# Autodesk Inventor assembly: 上層部
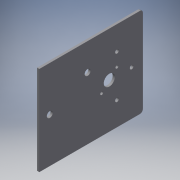
[picture p0: Inventor's stored thumbnail of the model, 180x180]
Saved by Autodesk Inventor 2019 (Build 230136000, 136)
## iProperties
Created: 2020-10-06
Part Number: 上層部
Material: 一般
Document SubType Name: Assembly
Designer: zhept
Author: zhept
## Documents named in this file (2)
- C:\Users\zhept\OneDrive\大学\rrst\足回り2020\上層部.iam
- C:\Users\zhept\OneDrive\大学\rrst\足回り2020\足回り試作　ゴム車輪\板.ipt
## Components (1 placed, 1 different names)
1. 板:1 — メイト:1, 角度:1
## Relationships (2: Mate 1, Angle 1)
- メイト:1 [Mate]: 板:1
- 角度:1 [Angle] (0 deg): 板:1
